# Autodesk Inventor assembly: MGN7 Rail (2)
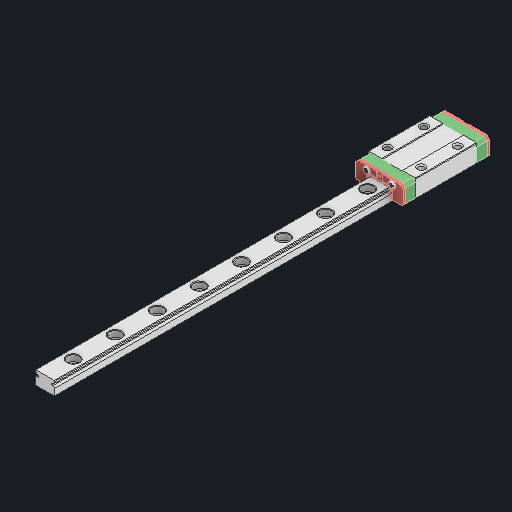
[picture p0: Inventor's stored thumbnail of the model, 512x512]
Saved by Autodesk Inventor 2025.1 (Build 291241020, 241B)
## iProperties
Created: 2025-05-09
Part Number: MGN7 Rail (2)
Document SubType Name: Assembly
Designer: AdminForWorker
Title: MGN7 Rail 150mm
Author: AdminForWorker
## Documents named in this file (4)
- C:\Users\Joshua Eah\Documents\Voron 0.2\CAD\Master Assembly\MGN7 Rail (2).iam
- MGN7 Rail 150mm.iam
- C:\Users\Joshua Eah\Documents\Voron 0.2\CAD\Master Assembly\Part44.ipt
- C:\Users\Joshua Eah\Documents\Voron 0.2\CAD\Master Assembly\MGN7H Carriage.ipt
## Components (2 placed, 2 different names)
1. MGN7H Carriage:1 — Cylindrical:1, Cylindrical:2
2. 150mm Rail — Cylindrical:1, Cylindrical:2
## Relationships (2: CylindricalJoint 2)
- Cylindrical:1: MGN7H Carriage:1 ↔ 150mm Rail
- Cylindrical:2: MGN7H Carriage:1 ↔ 150mm Rail
